# Autodesk Inventor assembly: AM14U3 Wide Frame Half
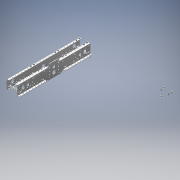
[picture p0: Inventor's stored thumbnail of the model, 180x180]
Saved by Autodesk Inventor 2017 (Build 210142000, 142)
## iProperties
Created: 2017-01-12
Part Number: AM14U3 Wide Frame Half
Document SubType Name: Assembly
Designer: Ben
Author: Ben
Revision Number: ANY
## Documents named in this file (5)
- C:\Users\Ben\Desktop\Projects\2017 Robot\Frame\AM14U3 Wide Frame Half.iam
- C:\Users\Ben\Desktop\Projects\2017 Robot\Frame\Churro 3375.ipt
- C:\Users\Ben\Desktop\Projects\2017 Robot\Frame\FHTS 0.25-20-0.75_FHTS 0.25-20-G-0.75-C.ipt
- C:\Users\Ben\Desktop\Projects\2017 Robot\Frame\AM14U3 Outside Sheet Wide.ipt
- C:\Users\Ben\Desktop\Projects\2017 Robot\Frame\AM14U3 Inside Sheet Wide.ipt
## Components (14 placed, 14 different names)
1. Churro 3375_53 — Mate:1
2. Churro 3375_54
3. Churro 3375_55
4. Churro 3375_56 — Insert:1
5. FHTS 0.25-20-0.75_FHTS 0.25-20-G-0.75-C_57
6. FHTS 0.25-20-0.75_FHTS 0.25-20-G-0.75-C_58
7. FHTS 0.25-20-0.75_FHTS 0.25-20-G-0.75-C_59
8. FHTS 0.25-20-0.75_FHTS 0.25-20-G-0.75-C_60
9. FHTS 0.25-20-0.75_FHTS 0.25-20-G-0.75-C_61
10. FHTS 0.25-20-0.75_FHTS 0.25-20-G-0.75-C_62
11. FHTS 0.25-20-0.75_FHTS 0.25-20-G-0.75-C_63
12. FHTS 0.25-20-0.75_FHTS 0.25-20-G-0.75-C_64
13. AM14U3 Outside Sheet Wide_101 — Mate:1, Flush:1, Flush:2
14. AM14U3 Inside Sheet Wide_102 — Flush:1, Flush:2, Insert:1
## Relationships (4: Flush 2, Mate 1, Insert 1)
- Mate:1: Churro 3375_53 ↔ AM14U3 Outside Sheet Wide_101
- Flush:1: AM14U3 Outside Sheet Wide_101 ↔ AM14U3 Inside Sheet Wide_102
- Flush:2: AM14U3 Outside Sheet Wide_101 ↔ AM14U3 Inside Sheet Wide_102
- Insert:1: Churro 3375_56 ↔ AM14U3 Inside Sheet Wide_102
